# Autodesk Inventor assembly: ChassisBase
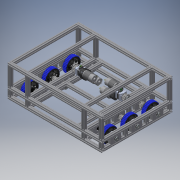
[picture p0: Inventor's stored thumbnail of the model, 180x180]
Saved by Autodesk Inventor 2018 (Build 220112000, 112)
## iProperties
Created: 2017-09-03
Part Number: ChassisBase
Document SubType Name: Assembly
Designer: snipe
Author: snipe
## Documents named in this file (13)
- E:\Clark\Assets\ClarkBody.iam
- E:\Clark\Assets\pro20in.ipt
- E:\Clark\Assets\pro36in.ipt
- E:\Clark\Assets\BearingBlock.ipt
- E:\Clark\Assets\DriveShaftA.iam
- E:\Clark\Assets\SideShaftA.iam
- E:\Clark\Assets\SideShaftB.iam
- E:\Clark\Assets\pro35mm.ipt
- E:\Clark\Assets\VPlan775dualinput.iam
- E:\Clark\Assets\24tPulley15mm.ipt
- E:\Clark\Assets\ShaftCollar.ipt
- E:\Clark\Assets\pro125mm.ipt
- E:\Clark\Assets\proWildStangin.ipt
## Components (70 placed, 25 different names)
1. VPlan775dualinput:1 [sub-assembly] — Flush:63, Mate:75, Mate:77, Mate:78, Mate:81, Mate:84, Mate:98, Mate:99
2. VPlan775dualinput:2 [sub-assembly] — Flush:64, Mate:76, Mate:79, Mate:80, Mate:82, Mate:96, Mate:100, Mate:101
3. 24tPulley15mm:1 — Mate:77, Mate:78, Mate:81, Flush:65, Mate:97
4. 24tPulley15mm:2 — Mate:79, Mate:80, Mate:82, Flush:66, Mate:95
5. ShaftCollar:1 — Mate:97, Mate:98, Mate:99
6. ShaftCollar:2 — Mate:95, Mate:96, Mate:100
7. pro125mm:1 — Mate:102, Flush:73, Flush:74, Mate:114, Flush:92, Mate:115
8. pro125mm:2 — Mate:103, Flush:75, Flush:76
9. pro125mm:3 — Mate:112, Flush:67, Flush:68
10. pro125mm:4 — Mate:111, Flush:69, Flush:70, Mate:116, Mate:117, Flush:93
11. pro125mm:5 — Mate:110, Flush:87, Flush:88, Mate:118, Flush:94, Mate:119
12. pro125mm:6 — Mate:109, Flush:85, Flush:86, Mate:120, Flush:95, Mate:121, Flush:99, Flush:101
13. pro125mm:7 — Mate:106, Flush:79, Flush:80, Flush:96, Flush:97
14. pro125mm:8 — Mate:105, Flush:77, Flush:78
15. pro36in:6 — Flush:99, Flush:100, Flush:101
16. pro36in:7 — Flush:96, Flush:97, Flush:98
17. pro20in:11 — Mate:116, Mate:117, Flush:93
18. pro20in:12 — Mate:118, Flush:94, Mate:119
19. pro20in:13 — Mate:114, Flush:92, Mate:115
20. pro20in:14 — Mate:120, Flush:95, Mate:121, Flush:98, Flush:100
21. proWildStangin:1 — Mate:124, Flush:103, Mate:125
22. proWildStangin:2 — Mate:122, Flush:102, Mate:123
23. pro36in:2 — Mate:1, Mate:2, Mate:3, Mate:4, Mate:5, Flush:1, Flush:2, Flush:3, Flush:4, Flush:5, Flush:6, Symmetry:1, Symmetry:2, Symmetry:3, Symmetry:4, Mate:48, Flush:26, Flush:27, Mate:52, Mate:59, Flush:48, Flush:49, Flush:51, Mate:60
24. pro20in:1 — Mate:2, Flush:5, Flush:6, Flush:7, Mate:8, Flush:8, Mate:31, Flush:19, Mate:32, Mate:33, Flush:20, Flush:21, Flush:23, Mate:46, Flush:24, Mate:47, Flush:25
25. pro20in:2 — Mate:5, Flush:1, Flush:2, Mate:9, Flush:9, Mate:11, Flush:10, Flush:11, Mate:20, Flush:15, Mate:55, Flush:40, Mate:58, Flush:47
26. pro20in:3 — Mate:3, Flush:4, Flush:16, Mate:28, Flush:17, Mate:29, Flush:18, Mate:30, Flush:28, Mate:50, Flush:30, Mate:51, Flush:32, Flush:35
27. pro20in:4 — Mate:4, Flush:3, Mate:15, Mate:16, Flush:12, Flush:13, Flush:14, Mate:19, Flush:15, Flush:39, Mate:56, Flush:42, Mate:57, Flush:45, Flush:52
28. pro36in:3 — Flush:7, Mate:8, Flush:8, Symmetry:1, Symmetry:2, Symmetry:3, Symmetry:4, Flush:22, Mate:45, Mate:49, Flush:29, Mate:53, Flush:36, Flush:37, Mate:54, Flush:38
29. DriveShaftA:1 [sub-assembly] — Mate:23, Mate:24, Flush:66, Mate:101
30. SideShaftA:1 [sub-assembly] — Mate:21, Mate:22, Mate:27
31. SideShaftB:1 [sub-assembly] — Mate:25, Mate:26
32. DriveShaftA:2 [sub-assembly] — Flush:65, Mate:84, Mate:85, Mate:92
33. SideShaftA:2 [sub-assembly] — Mate:86, Mate:87, Mate:90, Mate:91
34. SideShaftB:2 [sub-assembly] — Mate:88, Mate:93
35. RightBack — Mate:11, Flush:11, Mate:13
36. RightCenter — Flush:10, Mate:12, Mate:13, Mate:20
37. RightFront — Mate:9, Flush:9, Mate:12, Mate:27
38. RightBack2 — Mate:16, Flush:14, Mate:17, Mate:25, Mate:26
39. RightCenter2 — Flush:12, Mate:17, Mate:18, Mate:19, Mate:23, Mate:24
40. RightFront2 — Mate:15, Flush:13, Mate:18, Mate:21, Mate:22
41. LeftBack — Mate:32, Flush:21, Symmetry:5, Mate:86, Mate:87, Mate:89
42. LeftCenter — Mate:31, Flush:19, Mate:35, Symmetry:5, Symmetry:6, Mate:85, Mate:89, Mate:92
43. LeftFront — Mate:33, Flush:20, Mate:35, Symmetry:6, Mate:88, Mate:93
44. LeftBack2 — Flush:18, Mate:30, Mate:90, Mate:91
45. LeftCenter2 — Flush:17, Mate:29, Mate:94
46. LeftFront2 — Flush:16, Mate:28, Mate:94
47. pro35mm:13 — Mate:47, Flush:25, Flush:33, Flush:44, Flush:46, Flush:57
48. pro35mm:14 — Mate:46, Flush:24, Flush:31, Flush:41, Flush:43, Mate:63
49. pro35mm:15 — Mate:56, Flush:42, Flush:43, Mate:70
50. pro35mm:16 — Flush:44, Mate:57, Flush:45, Flush:60
51. pro35mm:17 — Mate:58, Flush:46, Flush:47, Mate:68, Flush:59
52. pro35mm:18 — Mate:55, Flush:40, Flush:41
53. pro35mm:3 — Mate:48, Flush:26, Flush:27, Flush:34
54. pro35mm:4 — Mate:52, Flush:34, Flush:35
55. pro35mm:5 — Flush:51, Mate:60, Flush:52
56. pro35mm:6 — Mate:59, Flush:48, Flush:49, Flush:55, Mate:62, Flush:56
57. pro35mm:8 — Mate:54, Flush:38, Flush:39
58. pro35mm:7 — Mate:53, Flush:36, Flush:37, Mate:61, Flush:53, Flush:54
59. pro35mm:11 — Mate:50, Flush:30, Flush:31, Mate:65, Flush:58
60. pro35mm:12 — Mate:51, Flush:32, Flush:33
61. pro35mm:2 — Mate:49, Flush:28, Flush:29
62. pro35mm:1 — Flush:22, Flush:23, Mate:45, Flush:73
63. proMidRight — Mate:73, Flush:62, Flush:64, Mate:76
64. proMidLeft — Mate:71, Flush:61, Flush:63, Mate:75, Mate:122, Flush:102, Mate:124, Flush:103
65. pro20in:5 — Mate:65, Flush:58, Mate:66, Flush:70, Flush:75
66. pro20in:6 — Mate:63, Flush:57, Mate:64, Flush:67, Flush:74
67. pro20in:7 — Mate:69, Mate:70, Flush:60, Flush:77, Flush:87
68. pro20in:8 — Mate:67, Mate:68, Flush:59
69. pro36in:4 — Flush:55, Mate:62, Flush:56, Mate:66, Mate:67, Mate:69, Mate:71, Flush:61, Mate:73, Flush:62, Mate:109, Mate:110, Mate:111, Mate:112, Flush:68, Flush:69, Flush:85, Flush:86, Flush:88
70. pro36in:5 — Mate:61, Flush:53, Flush:54, Mate:64, Mate:102, Mate:103, Mate:105, Mate:106, Flush:76, Flush:78, Flush:79, Flush:80, Mate:123, Mate:125
## Relationships (203: Mate 104, Flush 93, Symmetry 6)
- Mate:1: pro36in:2
- Mate:2: pro36in:2 ↔ pro20in:1
- Mate:3: pro36in:2 ↔ pro20in:3
- Mate:4: pro36in:2 ↔ pro20in:4
- Mate:5: pro36in:2 ↔ pro20in:2
- Flush:1: pro36in:2 ↔ pro20in:2
- Flush:2: pro36in:2 ↔ pro20in:2
- Flush:3: pro36in:2 ↔ pro20in:4
- Flush:4: pro36in:2 ↔ pro20in:3
- Flush:5: pro36in:2 ↔ pro20in:1
- Flush:6: pro36in:2 ↔ pro20in:1
- Flush:7: pro20in:1 ↔ pro36in:3
- Mate:8: pro20in:1 ↔ pro36in:3
- Flush:8: pro20in:1 ↔ pro36in:3
- Mate:9: pro20in:2 ↔ RightFront
- Flush:9: pro20in:2 ↔ RightFront
- Mate:11: pro20in:2 ↔ RightBack
- Flush:10: pro20in:2 ↔ RightCenter
- Flush:11: pro20in:2 ↔ RightBack
- Symmetry:1: pro36in:2 ↔ pro36in:3
- Mate:12 (147.447 mm): RightCenter ↔ RightFront
- Mate:13 (-147.447 mm): RightBack ↔ RightCenter
- Mate:15: pro20in:4 ↔ RightFront2
- Mate:16: pro20in:4 ↔ RightBack2
- Flush:12: pro20in:4 ↔ RightCenter2
- Flush:13: pro20in:4 ↔ RightFront2
- Flush:14: pro20in:4 ↔ RightBack2
- Symmetry:2: pro36in:2 ↔ pro36in:3
- Mate:17 (-147.447 mm): RightBack2 ↔ RightCenter2
- Mate:18 (147.447 mm): RightCenter2 ↔ RightFront2
- Mate:19: pro20in:4 ↔ RightCenter2
- Mate:20: pro20in:2 ↔ RightCenter
- Mate:21: SideShaftA:1 ↔ RightFront2
- Mate:22: SideShaftA:1 ↔ RightFront2
- Mate:23: DriveShaftA:1 ↔ RightCenter2
- Mate:24: DriveShaftA:1 ↔ RightCenter2
- Mate:25: SideShaftB:1 ↔ RightBack2
- Mate:26: SideShaftB:1 ↔ RightBack2
- Mate:27: SideShaftA:1 ↔ RightFront
- Flush:15: pro20in:2 ↔ pro20in:4
- Flush:16: pro20in:3 ↔ LeftFront2
- Mate:28: pro20in:3 ↔ LeftFront2
- Flush:17: pro20in:3 ↔ LeftCenter2
- Mate:29: pro20in:3 ↔ LeftCenter2
- Flush:18: pro20in:3 ↔ LeftBack2
- Mate:30: pro20in:3 ↔ LeftBack2
- Mate:31: pro20in:1 ↔ LeftCenter
- Flush:19: pro20in:1 ↔ LeftCenter
- Mate:32: pro20in:1 ↔ LeftBack
- Mate:33: pro20in:1 ↔ LeftFront
- Flush:20: pro20in:1 ↔ LeftFront
- Flush:21: pro20in:1 ↔ LeftBack
- Symmetry:3: pro36in:2 ↔ pro36in:3
- Symmetry:4: pro36in:2 ↔ pro36in:3
- Mate:35 (147.447 mm): LeftCenter ↔ LeftFront
- Flush:22: pro36in:3 ↔ pro35mm:1
- Flush:23: pro20in:1 ↔ pro35mm:1
- Mate:45: pro36in:3 ↔ pro35mm:1
- Mate:46: pro20in:1 ↔ pro35mm:14
- Flush:24: pro20in:1 ↔ pro35mm:14
- Symmetry:5: LeftBack ↔ LeftCenter
- Mate:47: pro20in:1 ↔ pro35mm:13
- Flush:25: pro20in:1 ↔ pro35mm:13
- Symmetry:6: LeftCenter ↔ LeftFront
- Mate:48: pro36in:2 ↔ pro35mm:3
- Flush:26: pro36in:2 ↔ pro35mm:3
- Flush:27: pro36in:2 ↔ pro35mm:3
- Mate:49: pro36in:3 ↔ pro35mm:2
- Flush:28: pro20in:3 ↔ pro35mm:2
- Flush:29: pro36in:3 ↔ pro35mm:2
- Mate:50: pro20in:3 ↔ pro35mm:11
- Flush:30: pro20in:3 ↔ pro35mm:11
- Flush:31: pro35mm:14 ↔ pro35mm:11
- Mate:51: pro20in:3 ↔ pro35mm:12
- Flush:32: pro20in:3 ↔ pro35mm:12
- Flush:33: pro35mm:13 ↔ pro35mm:12
- Mate:52: pro36in:2 ↔ pro35mm:4
- Flush:34: pro35mm:3 ↔ pro35mm:4
- Flush:35: pro20in:3 ↔ pro35mm:4
- Mate:53: pro36in:3 ↔ pro35mm:7
- Flush:36: pro36in:3 ↔ pro35mm:7
- Flush:37: pro36in:3 ↔ pro35mm:7
- Mate:54: pro36in:3 ↔ pro35mm:8
- Flush:38: pro36in:3 ↔ pro35mm:8
- Flush:39: pro20in:4 ↔ pro35mm:8
- Mate:55: pro20in:2 ↔ pro35mm:18
- Flush:40: pro20in:2 ↔ pro35mm:18
- Flush:41: pro35mm:14 ↔ pro35mm:18
- Mate:56: pro20in:4 ↔ pro35mm:15
- Flush:42: pro20in:4 ↔ pro35mm:15
- Flush:43: pro35mm:14 ↔ pro35mm:15
- Flush:44: pro35mm:13 ↔ pro35mm:16
- Mate:57: pro20in:4 ↔ pro35mm:16
- Flush:45: pro20in:4 ↔ pro35mm:16
- Mate:58: pro20in:2 ↔ pro35mm:17
- Flush:46: pro35mm:13 ↔ pro35mm:17
- Flush:47: pro20in:2 ↔ pro35mm:17
- Mate:59: pro36in:2 ↔ pro35mm:6
- Flush:48: pro36in:2 ↔ pro35mm:6
- Flush:49: pro36in:2 ↔ pro35mm:6
- Flush:51: pro36in:2 ↔ pro35mm:5
- Mate:60: pro36in:2 ↔ pro35mm:5
- Flush:52: pro20in:4 ↔ pro35mm:5
- Mate:61: pro35mm:7 ↔ pro36in:5
- Flush:53: pro35mm:7 ↔ pro36in:5
- Flush:54: pro35mm:7 ↔ pro36in:5
- Flush:55: pro35mm:6 ↔ pro36in:4
- Mate:62: pro35mm:6 ↔ pro36in:4
- Flush:56: pro35mm:6 ↔ pro36in:4
- Mate:63: pro35mm:14 ↔ pro20in:6
- Flush:57: pro35mm:13 ↔ pro20in:6
- Mate:64: pro20in:6 ↔ pro36in:5
- Mate:65: pro35mm:11 ↔ pro20in:5
- Flush:58: pro35mm:11 ↔ pro20in:5
- Mate:66: pro20in:5 ↔ pro36in:4
- Mate:67: pro20in:8 ↔ pro36in:4
- Mate:68: pro35mm:17 ↔ pro20in:8
- Flush:59: pro35mm:17 ↔ pro20in:8
- Mate:69: pro20in:7 ↔ pro36in:4
- Mate:70: pro35mm:15 ↔ pro20in:7
- Flush:60: pro35mm:16 ↔ pro20in:7
- Mate:71: proMidLeft ↔ pro36in:4
- Flush:61: proMidLeft ↔ pro36in:4
- Mate:73: proMidRight ↔ pro36in:4
- Flush:62: proMidRight ↔ pro36in:4
- Flush:63: VPlan775dualinput:1 ↔ proMidLeft
- Flush:64: VPlan775dualinput:2 ↔ proMidRight
- Mate:75: VPlan775dualinput:1 ↔ proMidLeft
- Mate:76: VPlan775dualinput:2 ↔ proMidRight
- Mate:77: VPlan775dualinput:1 ↔ 24tPulley15mm:1
- Mate:78: VPlan775dualinput:1 ↔ 24tPulley15mm:1
- Mate:79: VPlan775dualinput:2 ↔ 24tPulley15mm:2
- Mate:80: VPlan775dualinput:2 ↔ 24tPulley15mm:2
- Mate:81: VPlan775dualinput:1 ↔ 24tPulley15mm:1
- Mate:82: VPlan775dualinput:2 ↔ 24tPulley15mm:2
- Flush:65: 24tPulley15mm:1 ↔ DriveShaftA:2
- Flush:66: 24tPulley15mm:2 ↔ DriveShaftA:1
- Mate:84 (97.409 mm): VPlan775dualinput:1 ↔ DriveShaftA:2
- Mate:85: DriveShaftA:2 ↔ LeftCenter
- Mate:86: SideShaftA:2 ↔ LeftBack
- Mate:87: SideShaftA:2 ↔ LeftBack
- Mate:88: SideShaftB:2 ↔ LeftFront
- Mate:89 (147.447 mm): LeftBack ↔ LeftCenter
- Mate:90: SideShaftA:2 ↔ LeftBack2
- Mate:91: SideShaftA:2 ↔ LeftBack2
- Mate:92: DriveShaftA:2 ↔ LeftCenter
- Mate:93: SideShaftB:2 ↔ LeftFront
- Mate:94 (147.447 mm): LeftCenter2 ↔ LeftFront2
- Mate:95: 24tPulley15mm:2 ↔ ShaftCollar:2
- Mate:96: VPlan775dualinput:2 ↔ ShaftCollar:2
- Mate:97: 24tPulley15mm:1 ↔ ShaftCollar:1
- Mate:98: VPlan775dualinput:1 ↔ ShaftCollar:1
- Mate:99: VPlan775dualinput:1 ↔ ShaftCollar:1
- Mate:100: VPlan775dualinput:2 ↔ ShaftCollar:2
- Mate:101 (97.409 mm): VPlan775dualinput:2 ↔ DriveShaftA:1
- Mate:102: pro125mm:1 ↔ pro36in:5
- Mate:103: pro125mm:2 ↔ pro36in:5
- Mate:105: pro125mm:8 ↔ pro36in:5
- Mate:106: pro125mm:7 ↔ pro36in:5
- Mate:109: pro125mm:6 ↔ pro36in:4
- Mate:110: pro125mm:5 ↔ pro36in:4
- Mate:111: pro125mm:4 ↔ pro36in:4
- Mate:112: pro125mm:3 ↔ pro36in:4
- Flush:67: pro125mm:3 ↔ pro20in:6
- Flush:68: pro125mm:3 ↔ pro36in:4
- Flush:69: pro125mm:4 ↔ pro36in:4
- Flush:70: pro125mm:4 ↔ pro20in:5
- Flush:73: pro125mm:1 ↔ pro35mm:1
- Flush:74: pro125mm:1 ↔ pro20in:6
- Flush:75: pro125mm:2 ↔ pro20in:5
- Flush:76: pro125mm:2 ↔ pro36in:5
- Flush:77: pro125mm:8 ↔ pro20in:7
- Flush:78: pro125mm:8 ↔ pro36in:5
- Flush:79: pro125mm:7 ↔ pro36in:5
- Flush:80: pro125mm:7 ↔ pro36in:5
- Flush:85: pro125mm:6 ↔ pro36in:4
- Flush:86: pro125mm:6 ↔ pro36in:4
- Flush:87: pro125mm:5 ↔ pro20in:7
- Flush:88: pro125mm:5 ↔ pro36in:4
- Mate:114: pro125mm:1 ↔ pro20in:13
- Flush:92: pro125mm:1 ↔ pro20in:13
- Mate:115: pro125mm:1 ↔ pro20in:13
- Mate:116: pro125mm:4 ↔ pro20in:11
- Mate:117: pro125mm:4 ↔ pro20in:11
- Flush:93: pro125mm:4 ↔ pro20in:11
- Mate:118: pro125mm:5 ↔ pro20in:12
- Flush:94: pro125mm:5 ↔ pro20in:12
- Mate:119: pro125mm:5 ↔ pro20in:12
- Mate:120: pro125mm:6 ↔ pro20in:14
- Flush:95: pro125mm:6 ↔ pro20in:14
- Mate:121: pro125mm:6 ↔ pro20in:14
- Flush:96: pro125mm:7 ↔ pro36in:7
- Flush:97: pro125mm:7 ↔ pro36in:7
- Flush:98: pro36in:7 ↔ pro20in:14
- Flush:99: pro125mm:6 ↔ pro36in:6
- Flush:100: pro36in:6 ↔ pro20in:14
- Flush:101: pro125mm:6 ↔ pro36in:6
- Mate:122: proWildStangin:2 ↔ proMidLeft
- Flush:102: proWildStangin:2 ↔ proMidLeft
- Mate:123 (203.2 mm): proWildStangin:2 ↔ pro36in:5
- Mate:124: proWildStangin:1 ↔ proMidLeft
- Flush:103: proWildStangin:1 ↔ proMidLeft
- Mate:125 (101.6 mm): proWildStangin:1 ↔ pro36in:5
